# Autodesk Inventor assembly: structure
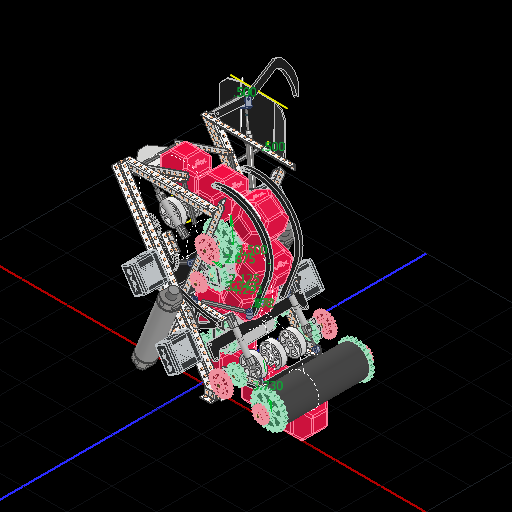
[picture p0: Inventor's stored thumbnail of the model, 512x512]
Saved by Autodesk Inventor 2025.2 (Build 292293000, 293)
## iProperties
Created: 2026-01-02
Part Number: structure
Document SubType Name: Assembly
Designer: cloudy
Author: cloudy
## Documents named in this file (50)
- C:\Users\cloudy\Documents\AURA_CAD\24\structure.iam
- C:\Users\cloudy\Documents\AURA_CAD\!lib\Electronics\V5 Simple Brain.ipt
- C:\Users\cloudy\Documents\AURA_CAD\!lib\Motion\Sprockets\9P Sprocket\9P 24T Sprocket, Square.iam
- C:\Users\cloudy\Documents\AURA_CAD\!lib\Motion\Wheels\Flex Wheels\2.000 Flex Wheel\2.000 30A .500.ipt
- C:\Users\cloudy\Documents\AURA_CAD\!lib\Structure\C Channel\Aluminum 1x3x1 Half\Alu C Half 1x3x1x7.ipt
- C:\Users\cloudy\Documents\AURA_CAD\15\30 stroke 10 bore\CJ2D10-30Z(0_0).iam
- C:\Users\cloudy\Documents\AURA_CAD\!lib\Motion\Shaft LS\Shaft Collar Metal\Shaft Collar No Screw.iam
- C:\Users\cloudy\Documents\AURA_CAD\!lib\Motion\Sprockets\9P Sprocket\9P 24T Sprocket, Circle.iam
- C:\Users\cloudy\Documents\AURA_CAD\!lib\Structure\C Channel\Aluminum 1x3x1 Half\Alu C Half 1x3x1x2.ipt
- C:\Users\cloudy\Documents\AURA_CAD\!lib\Structure\C Channel\Aluminum 1x3x1 Half Thick Cut\Alu C Half Thick 1x3x1x29.ipt
- C:\Users\cloudy\Documents\AURA_CAD\!lib\Structure\C Channel\Aluminum 1x2x1\Alu C 1x2x1x33.ipt
- C:\Users\cloudy\Documents\AURA_CAD\!lib\Structure\C Channel\Aluminum 1x3x1 Half\Alu C Half 1x3x1x11.ipt
- C:\Users\cloudy\Documents\AURA_CAD\!lib\Structure\C Channel\Aluminum 1x3x1 Half\Alu C Half 1x3x1x16.ipt
- C:\Users\cloudy\Documents\AURA_CAD\!lib\Structure\C Channel\Aluminum 1x3x1 Half\Alu C Half 1x3x1x15.ipt
- C:\Users\cloudy\Documents\AURA_CAD\24\centralbrace.ipt
- C:\Users\cloudy\Documents\AURA_CAD\!lib\Structure\Standoff\Standoff 1.00.ipt
- C:\Users\cloudy\Documents\AURA_CAD\!lib\Motion\Shaft LS\LS Pillow Bearing Block.ipt
- C:\Users\cloudy\Documents\AURA_CAD\!lib\Electronics\Motors with Screws\SteelM-StarS.iam
- C:\Users\cloudy\Documents\AURA_CAD\24\24t.ipt
- C:\Users\cloudy\Documents\AURA_CAD\24\40t.ipt
- C:\Users\cloudy\Documents\AURA_CAD\!lib\Motion\Insert Square.ipt
- C:\Users\cloudy\Documents\AURA_CAD\24\backalignermidgoal.ipt
- C:\Users\cloudy\Documents\AURA_CAD\!lib\Structure\Standoff\Standoff 3.00.ipt
- C:\Users\cloudy\Documents\AURA_CAD\!lib\Motion\Sprockets\9P Sprocket\9P 12T Sprocket, Circle.iam
- C:\Users\cloudy\Documents\AURA_CAD\!lib\Motion\Sprockets\6P Sprocket\6P 16T Sprocket, Circle.iam
- C:\Users\cloudy\Documents\AURA_CAD\!lib\Motion\Sprockets\6P Sprocket\6P 24T Sprocket, Circle.iam
- C:\Users\cloudy\Documents\AURA_CAD\!lib\Motion\Pneumatics\Legacy - SMC Pneumatics\Reservoir.ipt
- C:\Users\cloudy\Documents\AURA_CAD\24\roller 18t.iam
- C:\Users\cloudy\Documents\AURA_CAD\!lib\Game Objects\Push Back\cube.ipt
- C:\Users\cloudy\Documents\AURA_CAD\24\front rails.ipt
- C:\Users\cloudy\Documents\AURA_CAD\!lib\Structure\Standoff\Standoff .875.ipt
- C:\Users\cloudy\Documents\AURA_CAD\15\25 stroke 10 bore\CJ2D10-25Z(0_0).iam
- C:\Users\cloudy\Documents\AURA_CAD\!lib\Structure\C Channel\Aluminum 1x3x1 Half\Alu C Half 1x3x1x10.ipt
- C:\Users\cloudy\Documents\AURA_CAD\!lib\Structure\C Channel\Aluminum 1x3x1 Half\Alu C Half 1x3x1x3.ipt
- C:\Users\cloudy\Documents\AURA_CAD\24\hood.ipt
- C:\Users\cloudy\Documents\AURA_CAD\24\28t.ipt
- C:\Users\cloudy\Documents\AURA_CAD\24\42t.ipt
- C:\Users\cloudy\Documents\AURA_CAD\!lib\Motion\Pneumatics\Legacy - SMC Pneumatics\Double Acting Piston.iam
- C:\Users\cloudy\Documents\AURA_CAD\!lib\Motion\Pneumatics\Legacy - SMC Pneumatics\Cylinder Mount.ipt
- C:\Users\cloudy\Documents\AURA_CAD\24\wing.ipt
- C:\Users\cloudy\Documents\AURA_CAD\24\aligner.ipt
- C:\Users\cloudy\Documents\AURA_CAD\24\intakeroller.ipt
- C:\Users\cloudy\Documents\AURA_CAD\24\parkbrake.ipt
- C:\Users\cloudy\Documents\AURA_CAD\!lib\Motion\Wheels\Flex Wheels\2.000 Flex Wheel.ipt
- C:\Users\cloudy\Documents\AURA_CAD\!lib\Structure\Standoff.ipt
- C:\Users\cloudy\Documents\AURA_CAD\!lib\Electronics\Motors with Screws.iam
- C:\Users\cloudy\Documents\AURA_CAD\!lib\Motion\Shaft LS\Shaft Collar Metal.iam
- C:\Users\cloudy\Documents\AURA_CAD\!lib\Motion\Sprockets\9P Sprocket.iam
- C:\Users\cloudy\Documents\AURA_CAD\!lib\Motion\Sprockets\6P Sprocket.iam
- C:\Users\cloudy\Documents\AURA_CAD\24\Drivetrain\Wheels\Traction\brace.ipt
## Components (123 placed, 43 different names)
1. V5 Simple Brain:1 — Insert:17, Insert:18
2. 2.000 30A .500:2 — Insert:87
3. Alu C Half 1x3x1x7:1 — Insert:23, Mate:25, Insert:138, Flush:7
4. CJ2D10-30Z(0_0):1 [sub-assembly] — Insert:137, Mate:68
5. Alu C Half 1x3x1x2:5 — Insert:14
6. Alu C Half 1x3x1x2:6 — Insert:13
7. Alu C 1x2x1x33:1 — Insert:11, Insert:25, Insert:34, Insert:35, Insert:40, Insert:43, Insert:44, Mate:16, Insert:65, Insert:82, Insert:90, Mate:36, Mate:77, Insert:149, Mate:78, Insert:176, Mate:87, Insert:178, Mate:89
8. Alu C 1x2x1x33:2 — Insert:10, Insert:21, Insert:23, Insert:63, Insert:64, Insert:81, Insert:89, Mate:34, Insert:91, Mate:35, Mate:42, Insert:157, Insert:168, Insert:169, Insert:174, Insert:175, Insert:177, Mate:88
9. Alu C Half 1x3x1x2:7 — Insert:10
10. Alu C Half 1x3x1x2:8 — Insert:11
11. Alu C Half 1x3x1x11:1 — Insert:15, Insert:16, Insert:17, Insert:18
12. Alu C Half Thick 1x3x1x29:1 — Insert:13, Insert:15, Mate:9, Insert:49, Insert:102, Mate:38, Insert:109, Insert:110, Insert:147
13. Alu C Half Thick 1x3x1x29:2 — Insert:14, Insert:16, Mate:7, Insert:57, Insert:59, Insert:67, Mate:26, Insert:105, Insert:106
14. centralbrace:1 — Insert:21, Mate:7, Insert:46, Mate:18
15. centralbrace:2 — Insert:25, Mate:9, Insert:47, Mate:19
16. LS Pillow Bearing Block:1 — Insert:107, Insert:108, Insert:161
17. LS Pillow Bearing Block:2 — Insert:103, Insert:104, Insert:113, Insert:158
18. Standoff 1.00:5 — Insert:34
19. Standoff 1.00:6 — Insert:35
20. LS Pillow Bearing Block:3 — Insert:77, Insert:95
21. SteelM-StarS:3 [sub-assembly] — Insert:44, Mate:16
22. 24t:1 — Insert:38, Insert:39, Angle:1
23. 40t:1 — Insert:41, Insert:42, Angle:2
24. Insert Square:1 — Flush:2, Insert:42, Angle:2, Insert:43
25. Insert Square:2 — Flush:1, Insert:39, Insert:88
26. Insert Square:3 — Flush:1, Insert:38, Angle:1, Insert:40
27. Insert Square:4 — Flush:2, Insert:41
28. Alu C Half 1x3x1x15:1 — Insert:46, Mate:18, Insert:126, Insert:133
29. Alu C Half 1x3x1x15:2 — Insert:47, Mate:19, Flush:3, Mate:67, Mate:43, Insert:129
30. backalignermidgoal:1 — Flush:3, Insert:48, Insert:56, Insert:126, Mate:43
31. Shaft Collar No Screw:1 [sub-assembly] — Insert:48, Insert:51
32. Shaft Collar No Screw:2 [sub-assembly] — Insert:49, Insert:50
33. Shaft Collar No Screw:3 [sub-assembly] — Insert:50, Insert:52
34. Shaft Collar No Screw:4 [sub-assembly] — Insert:51, Mate:20
35. Standoff 3.00:7 — Insert:52, Mate:20
36. Shaft Collar No Screw:5 [sub-assembly] — Insert:56
37. Shaft Collar No Screw:6 [sub-assembly] — Insert:57
38. Shaft Collar No Screw:7 [sub-assembly] — Insert:58
39. Shaft Collar No Screw:8 [sub-assembly] — Mate:21
40. Standoff 3.00:8 — Insert:58, Mate:21
41. Alu C Half 1x3x1x16:2 — Insert:59, Mate:42
42. 9P 24T Sprocket, Circle:5 [sub-assembly] — Mate:31, Insert:93, Mate:85
43. 9P 24T Sprocket, Circle:6 [sub-assembly] — Mate:31, Insert:92, Mate:86
44. Standoff 1.00:9 — Insert:63
45. Standoff 1.00:10 — Insert:64
46. LS Pillow Bearing Block:4 — Insert:80, Insert:94
47. Alu C Half 1x3x1x7:2 — Insert:65, Mate:25, Insert:140
48. CJ2D10-30Z(0_0):2 [sub-assembly] — Mate:67, Insert:139, Mate:68
49. LS Pillow Bearing Block:5 — Insert:67, Mate:26
50. LS Pillow Bearing Block:6 — Insert:75, Insert:102, Mate:38, Insert:162
51. 9P 24T Sprocket, Square:9 [sub-assembly] — Insert:74, Insert:75
52. 9P 24T Sprocket, Square:10 [sub-assembly] — Insert:74
53. 2.000 30A .500:3 — Insert:83, Mate:39
54. 2.000 30A .500:4 — Insert:83, Insert:115
55. 9P 12T Sprocket, Circle:15 [sub-assembly] — Insert:82
56. 9P 12T Sprocket, Circle:16 [sub-assembly] — Insert:81, Insert:114
57. 6P 24T Sprocket, Circle:2 [sub-assembly] — Insert:77, Flush:6
58. 6P 24T Sprocket, Circle:3 [sub-assembly] — Insert:80, Flush:5
59. 2.000 30A .500:5 — Insert:86, Insert:87, Insert:88
60. 2.000 30A .500:6 — Insert:86
61. SteelM-StarS:6 [sub-assembly] — Insert:89, Mate:34
62. SteelM-StarS:7 [sub-assembly] — Insert:91, Mate:35
63. SteelM-StarS:8 [sub-assembly] — Insert:90, Mate:36
64. 9P 12T Sprocket, Circle:17 [sub-assembly] — Insert:94
65. 9P 12T Sprocket, Circle:18 [sub-assembly] — Insert:95, Mate:39
66. 6P 16T Sprocket, Circle:5 [sub-assembly] — Insert:93, Flush:6
67. 6P 16T Sprocket, Circle:6 [sub-assembly] — Insert:92, Flush:5
68. Reservoir:1
69. Reservoir:2
70. Standoff .875:11 — Insert:103, Insert:105
71. Standoff .875:12 — Insert:108, Insert:109
72. Standoff .875:13 — Insert:107, Insert:110
73. Standoff .875:14 — Insert:104, Insert:106
74. roller 18t:1 [sub-assembly] — Insert:114
75. roller 18t:2 [sub-assembly] — Insert:113
76. 2.000 30A .500:7 — Insert:115
77. cube:2
78. cube:3
79. cube:4
80. cube:5
81. cube:6
82. cube:7
83. cube:8
84. cube:9
85. cube:10
86. front rails:1 — Mate:44, Mate:46, Insert:130
87. front rails:2 — Mate:44, Mate:46, Insert:134
88. Shaft Collar No Screw:9 [sub-assembly] — Insert:130
89. Shaft Collar No Screw:10 [sub-assembly]
90. Shaft Collar No Screw:11 [sub-assembly] — Insert:129, Insert:135
91. Standoff 3.00:15 — Insert:135
92. Shaft Collar No Screw:12 [sub-assembly] — Insert:134
93. Shaft Collar No Screw:13 [sub-assembly]
94. Shaft Collar No Screw:14 [sub-assembly] — Insert:133, Mate:48, Insert:136
95. Standoff 3.00:16 — Mate:48, Insert:136
96. Shaft Collar No Screw:15 [sub-assembly] — Insert:137, Insert:138
97. Shaft Collar No Screw:16 [sub-assembly] — Insert:139, Insert:140
98. Shaft Collar No Screw:19 [sub-assembly]
99. CJ2D10-25Z(0_0):3 [sub-assembly] — Insert:145, Insert:150
100. Shaft Collar No Screw:21 [sub-assembly] — Insert:145, Mate:80
101. Alu C Half 1x3x1x16:3 — Insert:147, Mate:77, Insert:152
102. Alu C Half 1x3x1x3:1 — Insert:149, Mate:78, Insert:150
103. hood:1 — Insert:151, Mate:79, Insert:153, Mate:81
104. Standoff 3.00:17 — Insert:154
105. Alu C Half 1x3x1x10:1 — Insert:151, Mate:79, Mate:80, Insert:152, Insert:154, Insert:155
106. Alu C Half 1x3x1x10:2 — Insert:153, Mate:81, Insert:156
107. Standoff 3.00:18 — Insert:155
108. Standoff 3.00:19 — Insert:156
109. 28t:1 — Insert:158
110. 42t:1 — Insert:157
111. 6P 24T Sprocket, Circle:7 [sub-assembly] — Insert:162
112. 6P 16T Sprocket, Circle:10 [sub-assembly] — Insert:161
113. Double Acting Piston:1 [sub-assembly] — Insert:167, Insert:168
114. Cylinder Mount:1 — Insert:167, Mate:82
115. wing:1 — Insert:169, Mate:82
116. Standoff 3.00:22 — Insert:175
117. Standoff 3.00:23 — Insert:174
118. aligner:2
119. intakeroller:1 — Mate:85, Mate:86
120. Alu C Half 1x3x1x3:2 — Insert:176, Mate:87
121. Alu C Half 1x3x1x3:3 — Insert:177, Mate:88
122. parkbrake:1 — Flush:7
123. brace:1 — Insert:178, Mate:89
## Relationships (151: Insert 106, Mate 37, Flush 6, Angle 2)
- Insert:10 (12.7 mm): Alu C 1x2x1x33:2 ↔ Alu C Half 1x3x1x2:7
- Insert:11 (12.7 mm): Alu C 1x2x1x33:1 ↔ Alu C Half 1x3x1x2:8
- Insert:13: Alu C Half 1x3x1x2:6 ↔ Alu C Half Thick 1x3x1x29:1
- Insert:14: Alu C Half 1x3x1x2:5 ↔ Alu C Half Thick 1x3x1x29:2
- Insert:15: Alu C Half 1x3x1x11:1 ↔ Alu C Half Thick 1x3x1x29:1
- Insert:16: Alu C Half 1x3x1x11:1 ↔ Alu C Half Thick 1x3x1x29:2
- Insert:17 (3.175 mm): V5 Simple Brain:1 ↔ Alu C Half 1x3x1x11:1
- Insert:18 (3.175 mm): V5 Simple Brain:1 ↔ Alu C Half 1x3x1x11:1
- Insert:21: Alu C 1x2x1x33:2 ↔ centralbrace:1
- Mate:7: Alu C Half Thick 1x3x1x29:2 ↔ centralbrace:1
- Insert:23 (25.4 mm): Alu C Half 1x3x1x7:1 ↔ Alu C 1x2x1x33:2
- Insert:25: Alu C 1x2x1x33:1 ↔ centralbrace:2
- Mate:9: Alu C Half Thick 1x3x1x29:1 ↔ centralbrace:2
- [Insert]: Standoff 1.00:6 ↔ LS Pillow Bearing Block:3
- [Mate]: Standoff 1.00:5 ↔ LS Pillow Bearing Block:3
- Insert:34: Alu C 1x2x1x33:1 ↔ Standoff 1.00:5
- Insert:35: Alu C 1x2x1x33:1 ↔ Standoff 1.00:6
- Flush:1: Insert Square:2 ↔ Insert Square:3
- Insert:38: 24t:1 ↔ Insert Square:3
- Insert:39: 24t:1 ↔ Insert Square:2
- Angle:1 (0 deg): 24t:1 ↔ Insert Square:3
- Insert:40: Alu C 1x2x1x33:1 ↔ Insert Square:3
- Flush:2: Insert Square:1 ↔ Insert Square:4
- Insert:41: 40t:1 ↔ Insert Square:4
- Insert:42: 40t:1 ↔ Insert Square:1
- Angle:2 (0 deg): 40t:1 ↔ Insert Square:1
- Insert:43: Alu C 1x2x1x33:1 ↔ Insert Square:1
- Insert:44: Alu C 1x2x1x33:1 ↔ SteelM-StarS:3
- Mate:16: Alu C 1x2x1x33:1 ↔ SteelM-StarS:3
- Insert:46: centralbrace:1 ↔ Alu C Half 1x3x1x15:1
- Mate:18: centralbrace:1 ↔ Alu C Half 1x3x1x15:1
- Insert:47: centralbrace:2 ↔ Alu C Half 1x3x1x15:2
- Mate:19: centralbrace:2 ↔ Alu C Half 1x3x1x15:2
- Flush:3: Alu C Half 1x3x1x15:2 ↔ backalignermidgoal:1
- Insert:48: backalignermidgoal:1 ↔ Shaft Collar No Screw:1
- Insert:49: Alu C Half Thick 1x3x1x29:1 ↔ Shaft Collar No Screw:2
- Insert:50: Shaft Collar No Screw:2 ↔ Shaft Collar No Screw:3
- Insert:51: Shaft Collar No Screw:1 ↔ Shaft Collar No Screw:4
- Insert:52: Shaft Collar No Screw:3 ↔ Standoff 3.00:7
- Mate:20: Shaft Collar No Screw:4 ↔ Standoff 3.00:7
- [Insert]: Shaft Collar No Screw:6 ↔ Shaft Collar No Screw:7
- [Insert]: Shaft Collar No Screw:5 ↔ Shaft Collar No Screw:8
- Insert:56: backalignermidgoal:1 ↔ Shaft Collar No Screw:5
- Insert:57: Alu C Half Thick 1x3x1x29:2 ↔ Shaft Collar No Screw:6
- Insert:58: Shaft Collar No Screw:7 ↔ Standoff 3.00:8
- Mate:21: Shaft Collar No Screw:8 ↔ Standoff 3.00:8
- Insert:59 (22.225 mm): Alu C Half Thick 1x3x1x29:2 ↔ Alu C Half 1x3x1x16:2
- [Insert]: Standoff 1.00:10 ↔ LS Pillow Bearing Block:4
- [Mate]: Standoff 1.00:9 ↔ LS Pillow Bearing Block:4
- Insert:63: Alu C 1x2x1x33:2 ↔ Standoff 1.00:9
- Insert:64: Alu C 1x2x1x33:2 ↔ Standoff 1.00:10
- Insert:65 (25.4 mm): Alu C 1x2x1x33:1 ↔ Alu C Half 1x3x1x7:2
- Mate:25: Alu C Half 1x3x1x7:1 ↔ Alu C Half 1x3x1x7:2
- Mate:67: Alu C Half 1x3x1x15:2 ↔ CJ2D10-30Z(0_0):2
- Insert:67 (12.7 mm): Alu C Half Thick 1x3x1x29:2 ↔ LS Pillow Bearing Block:5
- Mate:26: Alu C Half Thick 1x3x1x29:2 ↔ LS Pillow Bearing Block:5
- Insert:74 (82.55 mm): 9P 24T Sprocket, Square:9 ↔ 9P 24T Sprocket, Square:10
- Insert:75 (6.35 mm): LS Pillow Bearing Block:6 ↔ 9P 24T Sprocket, Square:9
- Insert:77 (6.35 mm): LS Pillow Bearing Block:3 ↔ 6P 24T Sprocket, Circle:2
- Insert:80 (6.35 mm): LS Pillow Bearing Block:4 ↔ 6P 24T Sprocket, Circle:3
- Insert:81 (4.7625 mm): Alu C 1x2x1x33:2 ↔ 9P 12T Sprocket, Circle:16
- Insert:82 (4.7625 mm): Alu C 1x2x1x33:1 ↔ 9P 12T Sprocket, Circle:15
- Insert:83 (31.75 mm): 2.000 30A .500:3 ↔ 2.000 30A .500:4
- Insert:86 (69.85 mm): 2.000 30A .500:5 ↔ 2.000 30A .500:6
- Insert:87 (28.575 mm): 2.000 30A .500:2 ↔ 2.000 30A .500:5
- Insert:88 (36.449 mm): Insert Square:2 ↔ 2.000 30A .500:5
- Mate:31: 9P 24T Sprocket, Circle:5 ↔ 9P 24T Sprocket, Circle:6
- Insert:89: Alu C 1x2x1x33:2 ↔ SteelM-StarS:6
- Mate:34: Alu C 1x2x1x33:2 ↔ SteelM-StarS:6
- Insert:90: Alu C 1x2x1x33:1 ↔ SteelM-StarS:8
- Insert:91: Alu C 1x2x1x33:2 ↔ SteelM-StarS:7
- Mate:35: Alu C 1x2x1x33:2 ↔ SteelM-StarS:7
- Mate:36: Alu C 1x2x1x33:1 ↔ SteelM-StarS:8
- Insert:92 (6.35 mm): 9P 24T Sprocket, Circle:6 ↔ 6P 16T Sprocket, Circle:6
- Insert:93 (6.35 mm): 9P 24T Sprocket, Circle:5 ↔ 6P 16T Sprocket, Circle:5
- Flush:5: 6P 24T Sprocket, Circle:3 ↔ 6P 16T Sprocket, Circle:6
- Flush:6: 6P 24T Sprocket, Circle:2 ↔ 6P 16T Sprocket, Circle:5
- Insert:94 (9.525 mm): LS Pillow Bearing Block:4 ↔ 9P 12T Sprocket, Circle:17
- Insert:95 (9.525 mm): LS Pillow Bearing Block:3 ↔ 9P 12T Sprocket, Circle:18
- Insert:102 (12.7 mm): Alu C Half Thick 1x3x1x29:1 ↔ LS Pillow Bearing Block:6
- Mate:38: Alu C Half Thick 1x3x1x29:1 ↔ LS Pillow Bearing Block:6
- Mate:39: 2.000 30A .500:3 ↔ 9P 12T Sprocket, Circle:18
- Insert:103: LS Pillow Bearing Block:2 ↔ Standoff .875:11
- Insert:104: LS Pillow Bearing Block:2 ↔ Standoff .875:14
- Insert:105: Alu C Half Thick 1x3x1x29:2 ↔ Standoff .875:11
- Insert:106: Alu C Half Thick 1x3x1x29:2 ↔ Standoff .875:14
- Insert:107: LS Pillow Bearing Block:1 ↔ Standoff .875:13
- Insert:108: LS Pillow Bearing Block:1 ↔ Standoff .875:12
- Insert:109: Alu C Half Thick 1x3x1x29:1 ↔ Standoff .875:12
- Insert:110: Alu C Half Thick 1x3x1x29:1 ↔ Standoff .875:13
- Insert:113 (6.35 mm): LS Pillow Bearing Block:2 ↔ roller 18t:2
- Insert:114 (23.495 mm): 9P 12T Sprocket, Circle:16 ↔ roller 18t:1
- Insert:115 (31.75 mm): 2.000 30A .500:4 ↔ 2.000 30A .500:7
- Mate:42: Alu C 1x2x1x33:2 ↔ Alu C Half 1x3x1x16:2
- Insert:126: Alu C Half 1x3x1x15:1 ↔ backalignermidgoal:1
- Mate:43: Alu C Half 1x3x1x15:2 ↔ backalignermidgoal:1
- Mate:44: front rails:1 ↔ front rails:2
- Mate:46: front rails:1 ↔ front rails:2
- [Insert]: Shaft Collar No Screw:9 ↔ Shaft Collar No Screw:10
- [Insert]: Shaft Collar No Screw:10 ↔ Standoff 3.00:15
- [Mate]: Shaft Collar No Screw:11 ↔ Standoff 3.00:15
- Insert:129: Alu C Half 1x3x1x15:2 ↔ Shaft Collar No Screw:11
- Insert:130: front rails:1 ↔ Shaft Collar No Screw:9
- [Insert]: Shaft Collar No Screw:12 ↔ Shaft Collar No Screw:13
- [Insert]: Shaft Collar No Screw:13 ↔ Standoff 3.00:16
- Insert:133: Alu C Half 1x3x1x15:1 ↔ Shaft Collar No Screw:14
- Insert:134: front rails:2 ↔ Shaft Collar No Screw:12
- Mate:48: Shaft Collar No Screw:14 ↔ Standoff 3.00:16
- Insert:135 (7 mm): Shaft Collar No Screw:11 ↔ Standoff 3.00:15
- Insert:136 (7 mm): Shaft Collar No Screw:14 ↔ Standoff 3.00:16
- Insert:137 (-2.54 mm): CJ2D10-30Z(0_0):1 ↔ Shaft Collar No Screw:15
- Insert:138: Alu C Half 1x3x1x7:1 ↔ Shaft Collar No Screw:15
- Insert:139 (-2.54 mm): CJ2D10-30Z(0_0):2 ↔ Shaft Collar No Screw:16
- Insert:140: Alu C Half 1x3x1x7:2 ↔ Shaft Collar No Screw:16
- Mate:68: CJ2D10-30Z(0_0):1 ↔ CJ2D10-30Z(0_0):2
- Insert:145 (-2.54 mm): CJ2D10-25Z(0_0):3 ↔ Shaft Collar No Screw:21
- Insert:147 (22.225 mm): Alu C Half Thick 1x3x1x29:1 ↔ Alu C Half 1x3x1x16:3
- Mate:77: Alu C 1x2x1x33:1 ↔ Alu C Half 1x3x1x16:3
- Insert:149 (25.4 mm): Alu C 1x2x1x33:1 ↔ Alu C Half 1x3x1x3:1
- Mate:78: Alu C 1x2x1x33:1 ↔ Alu C Half 1x3x1x3:1
- Insert:150 (19.05 mm): CJ2D10-25Z(0_0):3 ↔ Alu C Half 1x3x1x3:1
- Insert:151: hood:1 ↔ Alu C Half 1x3x1x10:1
- Mate:79: hood:1 ↔ Alu C Half 1x3x1x10:1
- Mate:80: Shaft Collar No Screw:21 ↔ Alu C Half 1x3x1x10:1
- Insert:152 (44.45 mm): Alu C Half 1x3x1x16:3 ↔ Alu C Half 1x3x1x10:1
- Insert:153: hood:1 ↔ Alu C Half 1x3x1x10:2
- Mate:81: hood:1 ↔ Alu C Half 1x3x1x10:2
- Insert:154 (6.35 mm): Standoff 3.00:17 ↔ Alu C Half 1x3x1x10:1
- Insert:155: Alu C Half 1x3x1x10:1 ↔ Standoff 3.00:18
- Insert:156: Alu C Half 1x3x1x10:2 ↔ Standoff 3.00:19
- Insert:157 (6.35 mm): Alu C 1x2x1x33:2 ↔ 42t:1
- Insert:158 (7.1437 mm): LS Pillow Bearing Block:2 ↔ 28t:1
- Insert:161 (6.35 mm): LS Pillow Bearing Block:1 ↔ 6P 16T Sprocket, Circle:10
- Insert:162 (6.35 mm): LS Pillow Bearing Block:6 ↔ 6P 24T Sprocket, Circle:7
- Insert:167 (-5 mm): Double Acting Piston:1 ↔ Cylinder Mount:1
- Insert:168: Alu C 1x2x1x33:2 ↔ Double Acting Piston:1
- Insert:169: Alu C 1x2x1x33:2 ↔ wing:1
- Mate:82: Cylinder Mount:1 ↔ wing:1
- [Insert] (19.05 mm): Standoff 3.00:22 ↔ aligner:2
- [Mate]: Standoff 3.00:23 ↔ aligner:2
- Insert:174: Alu C 1x2x1x33:2 ↔ Standoff 3.00:23
- Insert:175: Alu C 1x2x1x33:2 ↔ Standoff 3.00:22
- Mate:85: 9P 24T Sprocket, Circle:5 ↔ intakeroller:1
- Mate:86: 9P 24T Sprocket, Circle:6 ↔ intakeroller:1
- Insert:176 (6.35 mm): Alu C 1x2x1x33:1 ↔ Alu C Half 1x3x1x3:2
- Mate:87: Alu C 1x2x1x33:1 ↔ Alu C Half 1x3x1x3:2
- Insert:177 (6.35 mm): Alu C 1x2x1x33:2 ↔ Alu C Half 1x3x1x3:3
- Mate:88: Alu C 1x2x1x33:2 ↔ Alu C Half 1x3x1x3:3
- Flush:7: Alu C Half 1x3x1x7:1 ↔ parkbrake:1
- Insert:178 (19.05 mm): Alu C 1x2x1x33:1 ↔ brace:1
- Mate:89: Alu C 1x2x1x33:1 ↔ brace:1
## Named parameters: d70_d64 = 0 mm, d71_d65 = 0 mm, d107_d103 = 0 mm, d108_d104 = 0 mm, d126_d70_d64 = 0 mm, d127_d71_d65 = 0 mm, d237_d103 = 0 mm, d238_d105 = 0 mm, d239_d106 = 0 mm, d242_d237_d103 = 0 mm, d243_d238_d105 = 0 mm, d352_d350 = 19.05 mm, d353_d351 = 0 mm
